# Autodesk Inventor assembly: MG_996R
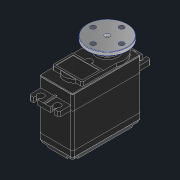
[picture p0: Inventor's stored thumbnail of the model, 180x180]
Saved by Autodesk Inventor 2021 (Build 250183000, 183)
## iProperties
Created: 2016-09-26
Part Number: MG_996R
Document SubType Name: Assembly
Designer: Julian
Mass: 36.0153 g
Surface Area: 118.599 cm^2
Volume: 31.6169 cm^3
Density: 1.13912 g/cm^3
Author: Julian
## Documents named in this file (6)
- C:\Users\yuta0\Downloads\新しいフォルダー\MG_996R.iam
- C:\Users\yuta0\Downloads\新しいフォルダー\servo_Base.ipt
- C:\Users\yuta0\Downloads\新しいフォルダー\Medio.ipt
- C:\Users\yuta0\Downloads\新しいフォルダー\Top.ipt
- C:\Users\yuta0\Downloads\新しいフォルダー\Eje.ipt
- C:\Users\yuta0\Documents\GitHub\catchrobo_hardware\catchrobo_robot\horn.ipt
## Components (5 placed, 5 different names)
1. Top:1 — De rotación:1, メイト:3, メイト:4, メイト:5, メイト:10, メイト:11
2. Medio:1 — メイト:3, メイト:4, メイト:5, メイト:6, メイト:7, メイト:8, 角度:2
3. servo_Base:1 — メイト:6, メイト:7, メイト:8
4. Eje:1 — De rotación:1
5. horn:1 — メイト:10, メイト:11, 角度:1
## Relationships (11: Mate 8, Angle 2, RevoluteJoint 1)
- De rotación:1 [RevoluteJoint]: Top:1 ↔ Eje:1
- メイト:3 [Mate]: Top:1 ↔ Medio:1
- メイト:4 [Mate]: Top:1 ↔ Medio:1
- メイト:5 [Mate]: Top:1 ↔ Medio:1
- メイト:6 [Mate]: Medio:1 ↔ servo_Base:1
- メイト:7 [Mate]: Medio:1 ↔ servo_Base:1
- メイト:8 [Mate]: Medio:1 ↔ servo_Base:1
- メイト:10 [Mate]: Top:1 ↔ horn:1
- メイト:11 [Mate]: Top:1 ↔ horn:1
- 角度:1 [Angle] (0 deg): horn:1
- 角度:2 [Angle] (0 deg): Medio:1
